# Autodesk Inventor assembly: A2017_T5_10
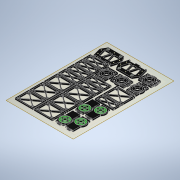
[picture p0: Inventor's stored thumbnail of the model, 180x180]
Saved by Autodesk Inventor 2022 (Build 260153000, 153)
## iProperties
Created: 2022-09-28
Part Number: A2017_T5_10
Document SubType Name: Assembly
Designer: Masato
Author: Masato
## Documents named in this file (7)
- C:\Users\MasatoKubotera\Documents\Inventor\SUSTAINA-OP\Cam\A2017_T5\A2017_T5_10.iam
- C:\Users\MasatoKubotera\Documents\Inventor\SUSTAINA-OP\Cam\DisposableBoard.ipt
- C:\Users\MasatoKubotera\Documents\Inventor\SUSTAINA-OP\LowerBody\Leg_joint\Leg_joint_yaw_frame.ipt
- C:\Users\MasatoKubotera\Documents\Inventor\SUSTAINA-OP\LowerBody\Link\BackLink_diagonal.ipt
- C:\Users\MasatoKubotera\Documents\Inventor\SUSTAINA-OP\LowerBody\Link\FrontLink_diagonal.ipt
- C:\Users\MasatoKubotera\Documents\Inventor\SUSTAINA-OP\UpperBody\UpperBody_horn_frame.ipt
- C:\Users\MasatoKubotera\Documents\Inventor\SUSTAINA-OP\UpperBody\Trunk\Trunk_lower_side_frame.ipt
## Components (25 placed, 6 different names)
1. DisposableBoard:1 — フラッシュ:1, フラッシュ:2, フラッシュ:3, フラッシュ:4, フラッシュ:5, フラッシュ:6
2. FrontLink_diagonal:1 — メイト:11, フラッシュ:11, メイト:15, 正接:5, フラッシュ:14, メイト:21
3. UpperBody_horn_frame:3 — メイト:20, フラッシュ:14, 正接:6
4. Trunk_lower_side_frame:1 — メイト:7, 正接:3, メイト:9, フラッシュ:10, メイト:10
5. Trunk_lower_side_frame:2 — メイト:8, フラッシュ:10, メイト:10
6. UpperBody_horn_frame:5 — メイト:17, 正接:5, メイト:21, 正接:6
7. UpperBody_horn_frame:6 — メイト:19, 正接:7, メイト:22, 正接:8, 正接:9, 角度:1
8. BackLink_diagonal:2 — メイト:12, メイト:13, 正接:4, フラッシュ:11, メイト:15
9. UpperBody_horn_frame:7 — メイト:18, 正接:8, 正接:9, 角度:1
10. FrontLink_diagonal:5 — メイト:1, フラッシュ:5, フラッシュ:6, フラッシュ:7, フラッシュ:9
11. FrontLink_diagonal:6
12. FrontLink_diagonal:7 — メイト:6
13. FrontLink_diagonal:8 — 正接:1
14. FrontLink_diagonal:9
15. FrontLink_diagonal:10 — フラッシュ:13, メイト:16
16. Leg_joint_yaw_frame:2 — フラッシュ:7, メイト:2, フラッシュ:8, 正接:1, 正接:2
17. Leg_joint_yaw_frame:4 — メイト:3, フラッシュ:8, 正接:2
18. Leg_joint_yaw_frame:5 — メイト:12
19. Leg_joint_yaw_frame:6 — 正接:4
20. BackLink_diagonal:7 — メイト:5, メイト:6, フラッシュ:9, 正接:3
21. BackLink_diagonal:8
22. BackLink_diagonal:9 — 正接:7
23. BackLink_diagonal:10 — メイト:9
24. BackLink_diagonal:11 — メイト:14, フラッシュ:13, メイト:16
25. BackLink_diagonal:12 — メイト:22
## Component patterns: (6 elements, first: FrontLink_diagonal:5), (2 elements, first: Leg_joint_yaw_frame:2 + Leg_joint_yaw_frame:4), (4 elements, first: BackLink_diagonal:7), (2 elements, first: BackLink_diagonal:11)
## Relationships (44: Mate 21, Flush 13, Tangent 9, Angle 1)
- フラッシュ:1 [Flush]: DisposableBoard:1
- フラッシュ:2 [Flush]: DisposableBoard:1
- フラッシュ:3 [Flush]: DisposableBoard:1
- フラッシュ:4 [Flush]: DisposableBoard:1
- メイト:1 [Mate]: FrontLink_diagonal:5
- フラッシュ:5 [Flush] (1.7 mm): DisposableBoard:1 ↔ FrontLink_diagonal:5
- フラッシュ:6 [Flush] (2 mm): DisposableBoard:1 ↔ FrontLink_diagonal:5
- フラッシュ:7 [Flush]: FrontLink_diagonal:5 ↔ Leg_joint_yaw_frame:2
- メイト:2 [Mate]: Leg_joint_yaw_frame:2
- メイト:3 [Mate]: Leg_joint_yaw_frame:4
- フラッシュ:8 [Flush]: Leg_joint_yaw_frame:2 ↔ Leg_joint_yaw_frame:4
- 正接:1 [Tangent] (2.1 mm): FrontLink_diagonal:8 ↔ Leg_joint_yaw_frame:2
- 正接:2 [Tangent] (2.1 mm): Leg_joint_yaw_frame:2 ↔ Leg_joint_yaw_frame:4
- メイト:5 [Mate]: BackLink_diagonal:7
- メイト:6 [Mate] (2.1 mm): FrontLink_diagonal:7 ↔ BackLink_diagonal:7
- フラッシュ:9 [Flush]: FrontLink_diagonal:5 ↔ BackLink_diagonal:7
- メイト:7 [Mate]: Trunk_lower_side_frame:1
- メイト:8 [Mate]: Trunk_lower_side_frame:2
- 正接:3 [Tangent]: Trunk_lower_side_frame:1 ↔ BackLink_diagonal:7
- メイト:9 [Mate] (2.1 mm): Trunk_lower_side_frame:1 ↔ BackLink_diagonal:10
- フラッシュ:10 [Flush]: Trunk_lower_side_frame:1 ↔ Trunk_lower_side_frame:2
- メイト:10 [Mate] (2.1 mm): Trunk_lower_side_frame:1 ↔ Trunk_lower_side_frame:2
- メイト:11 [Mate]: FrontLink_diagonal:1
- フラッシュ:11 [Flush]: FrontLink_diagonal:1 ↔ BackLink_diagonal:2
- メイト:15 [Mate] (2.1 mm): FrontLink_diagonal:1 ↔ BackLink_diagonal:2
- メイト:12 [Mate] (2.1 mm): BackLink_diagonal:2 ↔ Leg_joint_yaw_frame:5
- メイト:13 [Mate]: BackLink_diagonal:2
- 正接:4 [Tangent]: BackLink_diagonal:2 ↔ Leg_joint_yaw_frame:6
- メイト:14 [Mate]: BackLink_diagonal:11
- フラッシュ:13 [Flush]: FrontLink_diagonal:10 ↔ BackLink_diagonal:11
- メイト:16 [Mate] (2.1 mm): FrontLink_diagonal:10 ↔ BackLink_diagonal:11
- メイト:17 [Mate]: UpperBody_horn_frame:5
- メイト:18 [Mate]: UpperBody_horn_frame:7
- メイト:19 [Mate]: UpperBody_horn_frame:6
- メイト:20 [Mate]: UpperBody_horn_frame:3
- 正接:5 [Tangent]: FrontLink_diagonal:1 ↔ UpperBody_horn_frame:5
- フラッシュ:14 [Flush]: FrontLink_diagonal:1 ↔ UpperBody_horn_frame:3
- メイト:21 [Mate] (2.1 mm): FrontLink_diagonal:1 ↔ UpperBody_horn_frame:5
- 正接:6 [Tangent] (2.1 mm): UpperBody_horn_frame:3 ↔ UpperBody_horn_frame:5
- 正接:7 [Tangent] (2.1 mm): UpperBody_horn_frame:6 ↔ BackLink_diagonal:9
- メイト:22 [Mate] (2.1 mm): UpperBody_horn_frame:6 ↔ BackLink_diagonal:12
- 正接:8 [Tangent] (2.1 mm): UpperBody_horn_frame:6 ↔ UpperBody_horn_frame:7
- 正接:9 [Tangent]: UpperBody_horn_frame:6 ↔ UpperBody_horn_frame:7
- 角度:1 [Angle] (0 deg): UpperBody_horn_frame:6 ↔ UpperBody_horn_frame:7
